# Autodesk Inventor assembly: 193993 DSNU-40-300-P-A---(300PA---00--0-------0)
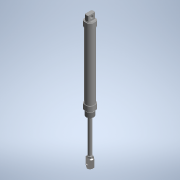
[picture p0: Inventor's stored thumbnail of the model, 180x180]
Saved by Autodesk Inventor 2022 (Build 260153000, 153)
## iProperties
Category: PARTsolutions
Company: FESTO
Part Number: 193993 DSNU-40-300-P-A---(300PA---00--0-------0)
Catalog Web Link: www.cadenas.de
Description: DSNU (m)-Round cylinder, Modular system
Vendor: FESTO
Document SubType Name: Assembly
Designer: partserver
Manufacturer: FESTO
Mass: 289.747 g
Surface Area: 1371.77 cm^2
Volume: 289.747 cm^3
Density: 1 g/cm^3
PSOL_IDENT_0: {ATYP=ASSISTANT},{DATA=script=$CADENAS_DATA/23d-libs/festo/webfesto.vbb/&M_FAMILY=DSNU&M_GROUP=01&M_
PSOL_IDENT_1: PARTNO=193993&IDCODE1=DSNU-40-300-P-A&IDCODE2=&C_DSNU_DM=40&C_DSNU_HEAD=DSNU&HUB=300&M_AA=A&M_DAA=P&
PSOL_IDENT_2: S_SMS=N&VCSD_UPDATE_YYIDENT11=DSNU-40-300-P-A&customer_number_cns=&MATES=1&LOD=HI&LOCKERP=1}
NB: 193993 DSNU-40-300-P-A---(300PA---00--0-------0)
NN: DSNU (m)
NT: Round cylinder, Modular system
NBSYN: $TNR. $IDCODE1.---($HUB.$DA.$PE.$ZD.$VS.$KA.$K2A.$K6.$K3.$K5.$K8.$KP.$R3.$R8.$TB.$KS.$LS.$ATEX.$HUBST.)
LINA: 193993 DSNU-40-300-P-A
CATALOG: Festo
OFFICIAL_STANDARD_NUMBERS: ISO 6432
TNR: 193993
TYP: DSNU-40
KDM: 40
HUB: 300
HUBST: 0
DA: P
PE: A
ZD: -
VS: -
KA: -
K2A: 0
K6: 0
K3: -
K5: -
K8: 0
KP: -
R3: -
R8: -
TB: -
KS: -
LS: -
ATEX: -
A1: 35
A2: 500
A3: 8
A4: 70.5
AB: 38
AM: 24
B: 38
BB: 4
BE: M38x1,5
BS: 9
B1: 54
B2: 13
B3: 38
B4: 12
B5: 32
B6: 14
B7: 4
CD: 12
D: 46
D1: 38
D2: 16
D3: 41.6
D4: 12
D5: 42
D6: 50
D7: 38
EE: G1/4
EW: 18
F: 42
FF: M5
F1: 24
H: 48
H1: 7
KK: M12x1.25
K1: M8
K2: 3
KV: 0
KW: 10
KV2: 19
KW2: 6
L: 15
LH: 15
LK: 18
L1: 453.6
L2: 384.6
L3: 12
L4: 30
L5: 27
L6: 63
L7: 33
L8: 25
L9: 29
L10: 104.6
L11: 116.6
L12: 77.6
L13: 162.6
ST: 9
SW: 13
T: 12
WH: 39
X: 3.3
XC: 439.6
SUPPLIER: FESTO
ARTICLENO: 193993 DSNU-40-300-P-A---(300PA---00--0-------0)
BOMINFO: 193993 DSNU-40-300-P-A
CREATOR: CADENAS GmbH
Title: 193993 DSNU-40-300-P-A
Author: Cadenas PARTsolutions
Comments: Round cylinder, Modular system
## Documents named in this file (5)
- C:\Users\patri\OneDrive - Syddansk Universitet\2. Semester Master\Mekaniske Elementer\Mini Project\2020-10-23\Workspaces\Workspace\Stempel\193993 DSNU-40-300-P-A---(300PA---00--0-------0).iam
- C:\Users\patri\OneDrive - Syddansk Universitet\2. Semester Master\Mekaniske Elementer\Mini Project\2020-10-23\Workspaces\Workspace\Stempel\193993 DSNU-40-300-P---(A----0-ZR).ipt
- C:\Users\patri\OneDrive - Syddansk Universitet\2. Semester Master\Mekaniske Elementer\Mini Project\2020-10-23\Workspaces\Workspace\Stempel\193993 DSNU-40-300-P---(A---00--0-KS).ipt
- C:\Users\patri\OneDrive - Syddansk Universitet\2. Semester Master\Mekaniske Elementer\Mini Project\2020-10-23\Workspaces\Workspace\Stempel\IMS-01-001.ipt
- C:\Users\patri\OneDrive - Syddansk Universitet\2. Semester Master\Mekaniske Elementer\Mini Project\2020-10-23\Workspaces\Workspace\Stempel\DIN-439-B - M12x1_25(F).ipt
## Components (4 placed, 4 different names)
1. 193993 DSNU-40-300-P---(A----0-ZR):1 — Mate:7, Angle:2, Flush:1
2. 193993 DSNU-40-300-P---(A---00--0-KS):1 — Mate:3, Mate:7, Angle:2, Flush:1, Mate:8
3. IMS-01-001:1 — Mate:3, Insert:1
4. DIN-439-B - M12x1_25(F):1 — Insert:1, Mate:8
## Relationships (6: Mate 3, Angle 1, Flush 1, Insert 1)
- Mate:3: 193993 DSNU-40-300-P---(A---00--0-KS):1 ↔ IMS-01-001:1
- Mate:7: 193993 DSNU-40-300-P---(A----0-ZR):1 ↔ 193993 DSNU-40-300-P---(A---00--0-KS):1
- Angle:2 (0 deg): 193993 DSNU-40-300-P---(A----0-ZR):1 ↔ 193993 DSNU-40-300-P---(A---00--0-KS):1
- Flush:1 (33 mm): 193993 DSNU-40-300-P---(A----0-ZR):1 ↔ 193993 DSNU-40-300-P---(A---00--0-KS):1
- Insert:1: IMS-01-001:1 ↔ DIN-439-B - M12x1_25(F):1
- Mate:8 (2 mm): 193993 DSNU-40-300-P---(A---00--0-KS):1 ↔ DIN-439-B - M12x1_25(F):1
